# Autodesk Inventor assembly: 393 Motor Casing
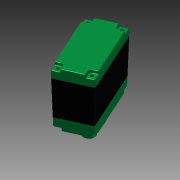
[picture p0: Inventor's stored thumbnail of the model, 180x180]
Saved by Autodesk Inventor 2015 (Build 190159000, 159)
## iProperties
Created: 2016-09-21
Part Number: 393 Motor Casing
Document SubType Name: Assembly
Designer: L
Author: IFI
Title: 276-2177 Rev1.STEP
Organization: IFI
Description: STEP AP203
Creation Date: 2010-06-25
Sending System: SolidWorks 2009
Preprocessor: SwSTEP 2.0
Author: L
## Documents named in this file (6)
- C:\Users\Leo\Google Drive\StarStuckProject\Starstruck\VEX Parts\Electronics\Compulsory\393 Motor Casing.iam
- C:\Users\Leo\Google Drive\StarStuckProject\Starstruck\Imported Components\393 Motor\276-2177-002 Rev1.ipt
- C:\Users\Leo\Google Drive\StarStuckProject\Starstruck\Imported Components\393 Motor\276-2177-001 Rev1.ipt
- C:\Users\Leo\Google Drive\StarStuckProject\Starstruck\Imported Components\393 Motor\276-2177-003 Rev1.ipt
- C:\Users\Leo\Google Drive\StarStuckProject\Starstruck\Imported Components\393 Motor\276-2177-008 Rev1.ipt
- C:\Users\Leo\Google Drive\StarStuckProject\Starstruck\Imported Components\393 Motor\276-2177-019 Rev1.ipt
## Components (6 placed, 5 different names)
1. 276-2177-002 Rev1_4 — Mate:1, Mate:2, Mate:3, Mate:4, Tangent:1, Tangent:2, Mate:5
2. 276-2177-001 Rev1_8 — Mate:1, Mate:2, Mate:3
3. 276-2177-003 Rev1_26 — Mate:4, Tangent:1, Tangent:2, Tangent:3, Mate:6, Mate:7, Tangent:4, Tangent:5, Tangent:6, Tangent:7
4. 276-2177-008 Rev1:1 — Mate:5, Tangent:3
5. 276-2177-019 Rev1:1 — Mate:7, Tangent:4, Tangent:7
6. 276-2177-019 Rev1:2 — Mate:6, Tangent:5, Tangent:6
## Relationships (14: Mate 7, Tangent 7)
- Mate:1: 276-2177-002 Rev1_4 ↔ 276-2177-001 Rev1_8
- Mate:2: 276-2177-002 Rev1_4 ↔ 276-2177-001 Rev1_8
- Mate:3: 276-2177-002 Rev1_4 ↔ 276-2177-001 Rev1_8
- Mate:4: 276-2177-002 Rev1_4 ↔ 276-2177-003 Rev1_26
- Tangent:1 (-1.9 mm): 276-2177-002 Rev1_4 ↔ 276-2177-003 Rev1_26
- Tangent:2 (-1.9 mm): 276-2177-002 Rev1_4 ↔ 276-2177-003 Rev1_26
- Mate:5: 276-2177-002 Rev1_4 ↔ 276-2177-008 Rev1:1
- Tangent:3: 276-2177-003 Rev1_26 ↔ 276-2177-008 Rev1:1
- Mate:6: 276-2177-003 Rev1_26 ↔ 276-2177-019 Rev1:2
- Mate:7: 276-2177-003 Rev1_26 ↔ 276-2177-019 Rev1:1
- Tangent:4: 276-2177-003 Rev1_26 ↔ 276-2177-019 Rev1:1
- Tangent:5: 276-2177-003 Rev1_26 ↔ 276-2177-019 Rev1:2
- Tangent:6: 276-2177-003 Rev1_26 ↔ 276-2177-019 Rev1:2
- Tangent:7: 276-2177-003 Rev1_26 ↔ 276-2177-019 Rev1:1
